# Autodesk Inventor assembly: Pata - Ensamble_Lado_Izq
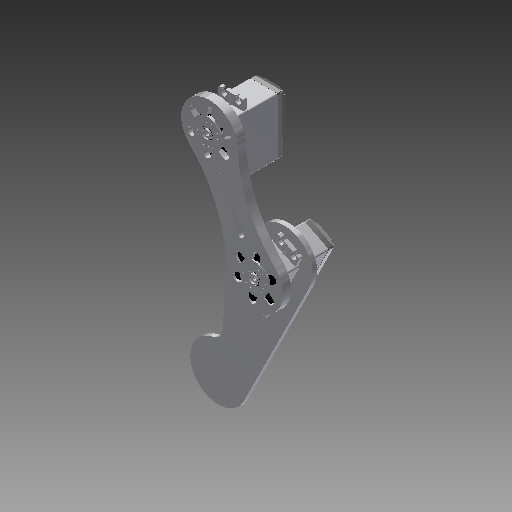
[picture p0: Inventor's stored thumbnail of the model, 512x512]
Saved by Autodesk Inventor 2019 (Build 230136000, 136)
## iProperties
Created: 2020-02-12
Part Number: Pata - Ensamble_Lado_Izq
Document SubType Name: Assembly
Designer: jacqu
Mass: 47.369 g
Surface Area: 327.582 cm^2
Volume: 47.369 cm^3
Density: 1 g/cm^3
Author: jacqu
## Documents named in this file (4)
- C:\Users\jacqu\Desktop\Robotica1_Proyecto-Cuadrupedo-master\Robotica1-Proyecto_Cuadrupedo\Pata - Ensamble_Lado_Izq.iam
- C:\Users\jacqu\Desktop\Robotica1_Proyecto-Cuadrupedo-master\Robotica1-Proyecto_Cuadrupedo\Pata - Antebrazo.ipt
- C:\Users\jacqu\Desktop\Robotica1_Proyecto-Cuadrupedo-master\Robotica1-Proyecto_Cuadrupedo\Pata - Brazo.ipt
- C:\Users\jacqu\Desktop\Robotica1_Proyecto-Cuadrupedo-master\Robotica1-Proyecto_Cuadrupedo\MG_996R.iam
## Components (4 placed, 3 different names)
1. Pata - Antebrazo:1 — Mate:5, Mate:6, Mate:7, Mate:8
2. Pata - Brazo:1 — Mate:9, Mate:10, Mate:11
3. MG_996R:1 [sub-assembly] — Mate:5, Mate:8, Mate:9, Mate:10, Mate:11
4. MG_996R:2 [sub-assembly] — Mate:6, Mate:7
## Relationships (7: Mate 7)
- Mate:5: Pata - Antebrazo:1 ↔ MG_996R:1
- Mate:6: Pata - Antebrazo:1 ↔ MG_996R:2
- Mate:7: Pata - Antebrazo:1 ↔ MG_996R:2
- Mate:8: Pata - Antebrazo:1 ↔ MG_996R:1
- Mate:9: Pata - Brazo:1 ↔ MG_996R:1
- Mate:10: Pata - Brazo:1 ↔ MG_996R:1
- Mate:11: Pata - Brazo:1 ↔ MG_996R:1
